# Autodesk Inventor assembly: Lucotte BOX
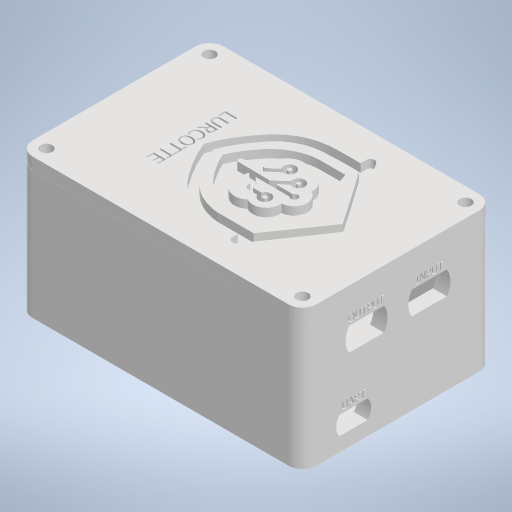
[picture p0: Inventor's stored thumbnail of the model, 512x512]
Saved by Autodesk Inventor 2024 (Build 280153000, 153)
## iProperties
Created: 2025-05-18
Part Number: Lucotte BOX
Document SubType Name: Assembly
Designer: chaaa
Author: chaaa
## Documents named in this file (3)
- C:\PENS\Semester 4\Mikrokontroller\Final Project\Mekanik\Lucotte BOX.iam
- C:\PENS\Semester 4\Mikrokontroller\Final Project\Mekanik\BOX Lurcotte.ipt
- C:\PENS\Semester 4\Mikrokontroller\Final Project\Mekanik\Cover Lurcotte.ipt
## Components (2 placed, 2 different names)
1. BOX Lurcotte:1 — Flush:1, Mate:1
2. Cover Lurcotte:1 — Flush:1, Mate:1
## Relationships (2: Flush 1, Mate 1)
- Flush:1 (-5 mm): BOX Lurcotte:1 ↔ Cover Lurcotte:1
- Mate:1: BOX Lurcotte:1 ↔ Cover Lurcotte:1
